# Autodesk Inventor assembly: Shelf
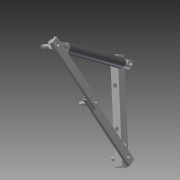
[picture p0: Inventor's stored thumbnail of the model, 180x180]
Saved by Autodesk Inventor 2013 (Build 170138000, 138)
## iProperties
Created: 2014-05-22
Part Number: Shelf
Document SubType Name: Assembly
Designer: nojessen
Mass: 1814.18 g
Surface Area: 1704.03 cm^2
Volume: 260.377 cm^3
Density: 6.9675 g/cm^3
Author: nojessen
## Documents named in this file (9)
- C:\Users\nojessen\Documents\GitHub\IED_Virtual_Design_Challenge\CAD\Shelf.iam
- C:\Users\nojessen\Documents\GitHub\IED_Virtual_Design_Challenge\CAD\Clip for Pin.ipt
- C:\Users\nojessen\Documents\GitHub\IED_Virtual_Design_Challenge\CAD\Horizantal Rod.ipt
- C:\Users\nojessen\Documents\GitHub\IED_Virtual_Design_Challenge\CAD\Pin.ipt
- C:\Users\nojessen\Documents\GitHub\IED_Virtual_Design_Challenge\CAD\Vertical Rod.ipt
- C:\Users\nojessen\Documents\GitHub\IED_Virtual_Design_Challenge\CAD\Piece One-Diagonal Piece.ipt
- C:\Users\nojessen\Documents\GitHub\IED_Virtual_Design_Challenge\CAD\Piece Two-Diagonal Piece.ipt
- C:\Users\nojessen\Documents\GitHub\IED_Virtual_Design_Challenge\CAD\Sleeve.ipt
- C:\Users\nojessen\Documents\GitHub\IED_Virtual_Design_Challenge\CAD\LongPin.ipt
## Components (14 placed, 8 different names)
1. Clip for Pin:1
2. Vertical Rod:1 — Mate:4, Mate:5, Mate:12, Flush:3
3. Pin:1 — Mate:8, Mate:9, Mate:19
4. Pin:2 — Mate:16, Mate:17, Mate:18
5. Pin:3 — Mate:10, Mate:11, Mate:20
6. Piece One-Diagonal Piece:1 — Mate:6, Mate:7, Flush:1, Mate:8, Mate:9, Mate:13, Mate:14, Mate:16, Mate:17
7. Piece Two-Diagonal Piece:1 — Mate:4, Mate:5, Mate:6, Mate:7, Flush:1, Mate:10, Mate:11
8. Horizantal Rod:1 — Mate:12, Mate:13, Mate:14, Mate:15, Flush:2, Mate:21
9. Sleeve:1 — Mate:15, Flush:2
10. Clip for Pin:2 — Mate:20
11. Clip for Pin:3 — Mate:19
12. Clip for Pin:4 — Mate:18
13. Clip for Pin:5 — Mate:22
14. LongPin:1 — Mate:21, Flush:3, Mate:22
## Relationships (22: Mate 19, Flush 3)
- Mate:4: Vertical Rod:1 ↔ Piece Two-Diagonal Piece:1
- Mate:5: Vertical Rod:1 ↔ Piece Two-Diagonal Piece:1
- Mate:6: Piece One-Diagonal Piece:1 ↔ Piece Two-Diagonal Piece:1
- Mate:7: Piece One-Diagonal Piece:1 ↔ Piece Two-Diagonal Piece:1
- Flush:1: Piece One-Diagonal Piece:1 ↔ Piece Two-Diagonal Piece:1
- Mate:8: Pin:1 ↔ Piece One-Diagonal Piece:1
- Mate:9: Pin:1 ↔ Piece One-Diagonal Piece:1
- Mate:10: Pin:3 ↔ Piece Two-Diagonal Piece:1
- Mate:11: Pin:3 ↔ Piece Two-Diagonal Piece:1
- Mate:12: Vertical Rod:1 ↔ Horizantal Rod:1
- Mate:13: Piece One-Diagonal Piece:1 ↔ Horizantal Rod:1
- Mate:14: Piece One-Diagonal Piece:1 ↔ Horizantal Rod:1
- Mate:15: Horizantal Rod:1 ↔ Sleeve:1
- Flush:2 (25.4 mm): Horizantal Rod:1 ↔ Sleeve:1
- Mate:16: Pin:2 ↔ Piece One-Diagonal Piece:1
- Mate:17: Pin:2 ↔ Piece One-Diagonal Piece:1
- Mate:18: Pin:2 ↔ Clip for Pin:4
- Mate:19: Pin:1 ↔ Clip for Pin:3
- Mate:20: Pin:3 ↔ Clip for Pin:2
- Mate:21: Horizantal Rod:1 ↔ LongPin:1
- Flush:3 (-30.48 mm): Vertical Rod:1 ↔ LongPin:1
- Mate:22: Clip for Pin:5 ↔ LongPin:1
